# Autodesk Inventor assembly: アームアセンブリ
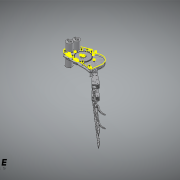
[picture p0: Inventor's stored thumbnail of the model, 180x180]
Saved by Autodesk Inventor 2020 (Build 240168000, 168)
## iProperties
Created: 2019-12-03
Part Number: アームアセンブリ
Material: 一般
Document SubType Name: Assembly
Designer: tanjihayato
Mass: 763.38 g
Surface Area: 1766.69 cm^2
Volume: 307.552 cm^3
Density: 2.48212 g/cm^3
Author: tanjihayato
## Documents named in this file (28)
- \\Mac\Home\Documents\Inventor\2019お遊び機体\アームアセンブリ.iam
- \\Mac\Home\Documents\Inventor\2019お遊び機体\アーム右フレーム.ipt
- \\Mac\Home\Documents\Inventor\2019お遊び機体\アーム真ん中フレーム.ipt
- \\Mac\Home\Documents\Inventor\2019お遊び機体\スペーサ　m3-l12.ipt
- \\Mac\Home\Documents\Inventor\2019お遊び機体\モーター(形だけ).ipt
- \\Mac\Home\Documents\Inventor\2019お遊び機体\キャップボルトM3×8.ipt
- \\Mac\Home\Documents\Inventor\2019お遊び機体\m1 64.ipt
- \\Mac\Home\Documents\Inventor\2019お遊び機体\m2z10はめあい.ipt
- \\Mac\Home\Documents\Inventor\2019お遊び機体\アーム左フレーム.ipt
- \\Mac\Home\Documents\Inventor\2019お遊び機体\スペーサ　m4-l35.ipt
- \\Mac\Home\Documents\Inventor\2019お遊び機体\スペーサ　m4-l18.ipt
- \\Mac\Home\Documents\Inventor\2019お遊び機体\アーム駆動抑え.ipt
- \\Mac\Home\Documents\Inventor\2019お遊び機体\フランジブッシュ　d6-D8-l5-h12.ipt
- \\Mac\Home\Documents\Inventor\2019お遊び機体\スペーサ　m3-l6.ipt
- \\Mac\Home\Documents\Inventor\2019お遊び機体\アーム最終段円盤.ipt
- \\Mac\Home\Documents\Inventor\2019お遊び機体\アーム中間節.ipt
- \\Mac\Home\Documents\Inventor\2019お遊び機体\アーム揺動節.ipt
- \\Mac\Home\Documents\Inventor\2019お遊び機体\アーム中間節_MIR.ipt
- \\Mac\Home\Documents\Inventor\2019お遊び機体\シールド殺し.ipt
- \\Mac\Home\Documents\Inventor\2019お遊び機体\ロッド.ipt
- \\Mac\Home\Documents\Inventor\2019お遊び機体\シールド殺し_MIR.ipt
- \\Mac\Home\Documents\Inventor\2019お遊び機体\ロッド根本.ipt
- \\Mac\Home\Documents\Inventor\2019お遊び機体\ロッド根本２.ipt
- \\Mac\Home\Documents\Inventor\2019お遊び機体\ロッド根本２_MIR.ipt
- \\Mac\Home\Documents\Inventor\2019お遊び機体\ロッド根本_MIR.ipt
- \\Mac\Home\Documents\Inventor\2019お遊び機体\スペーサ　m3-l14.ipt
- \\Mac\Home\Documents\Inventor\2019お遊び機体\アダプター.ipt
- \\Mac\Home\Documents\Inventor\2019お遊び機体\アダプター_MIR.ipt
## Components (74 placed, 27 different names)
1. アーム右フレーム:1 — 挿入:10, メイト:1, 挿入:12, 挿入:14, 挿入:15, 挿入:16, 挿入:17, 挿入:18, 挿入:19, 挿入:20, 挿入:21, 挿入:22, 挿入:23, 挿入:33, 挿入:34, 挿入:35
2. アーム真ん中フレーム:1 — 挿入:1, 挿入:2, 挿入:3, 挿入:4, 挿入:5, 挿入:6, 挿入:7, 挿入:8, 挿入:9, 挿入:11, 挿入:13, 挿入:24, 挿入:25, 挿入:26, 挿入:27, 挿入:28, 挿入:29, 挿入:30, 挿入:31, 挿入:32, 挿入:37, 挿入:41
3. スペーサ　m3-l12:1 — 挿入:6
4. スペーサ　m3-l12:2 — 挿入:9
5. スペーサ　m3-l12:3 — 挿入:4, 挿入:10
6. スペーサ　m3-l12:4 — 挿入:8
7. スペーサ　m3-l12:5 — 挿入:5, メイト:1
8. スペーサ　m3-l12:6 — 挿入:7
9. スペーサ　m3-l12:7 — 挿入:1
10. スペーサ　m3-l12:8 — 挿入:3
11. スペーサ　m3-l12:9 — 挿入:2
12. モーター(形だけ):1 — 挿入:11
13. モーター(形だけ):2 — 挿入:14
14. モーター(形だけ):3 — 挿入:12
15. モーター(形だけ):4 — 挿入:13
16. キャップボルトM3×8:1 — 挿入:17
17. キャップボルトM3×8:2 — 挿入:15
18. キャップボルトM3×8:3 — 挿入:20
19. キャップボルトM3×8:4 — 挿入:18
20. キャップボルトM3×8:5 — 挿入:22
21. キャップボルトM3×8:6 — 挿入:19
22. キャップボルトM3×8:7 — 挿入:28
23. キャップボルトM3×8:8 — 挿入:27
24. キャップボルトM3×8:9 — 挿入:24
25. キャップボルトM3×8:10 — 挿入:25
26. キャップボルトM3×8:11 — 挿入:29
27. キャップボルトM3×8:12 — 挿入:26
28. キャップボルトM3×8:13 — 挿入:30
29. キャップボルトM3×8:14 — 挿入:23
30. キャップボルトM3×8:15 — 挿入:31
31. キャップボルトM3×8:16 — 挿入:21
32. キャップボルトM3×8:17 — 挿入:32
33. キャップボルトM3×8:18 — 挿入:16
34. m1 64:1 — フラッシュ:1, メイト:2, メイト:3
35. m2z10はめあい:1 — フラッシュ:1, メイト:2, メイト:3, 挿入:33
36. アーム左フレーム:1 — 挿入:36, メイト:4, 挿入:38
37. スペーサ　m4-l35:1 — 挿入:34, 挿入:36
38. スペーサ　m4-l35:2 — 挿入:35, メイト:4
39. スペーサ　m4-l18:1 — 挿入:37, メイト:7
40. アーム駆動抑え:1 — 挿入:39, メイト:5
41. フランジブッシュ　d6-D8-l5-h12:1 — 挿入:38, 挿入:40
42. スペーサ　m3-l6:1 — 挿入:39, 挿入:40
43. アーム最終段円盤:1 — 挿入:41, メイト:5, 挿入:44
44. アーム中間節:1 — 挿入:42, 挿入:43, メイト:6, 挿入:44, 挿入:73, メイト:20
45. アーム揺動節:1 — 挿入:42, メイト:7
46. アーム中間節_MIR:1 — 挿入:43, メイト:6, 挿入:74, メイト:21
47. シールド殺し:2 — 挿入:45, メイト:8
48. ロッド:1 — 挿入:46, メイト:9, 挿入:77, メイト:24, 挿入:79
49. ロッド:2 — 挿入:45, メイト:8, 挿入:76, メイト:23, 挿入:78
50. シールド殺し_MIR:1 — 挿入:46, メイト:9
51. ロッド根本:1 — 挿入:55, 挿入:56, 挿入:57, 挿入:72, メイト:19
52. ロッド根本２:1 — 挿入:54, 挿入:77, メイト:24
53. ロッド根本２:4 — 挿入:53, 挿入:76, メイト:23
54. ロッド根本:4 — 挿入:62, メイト:15
55. ロッド根本２_MIR:1 — 挿入:51, 挿入:67, 挿入:68, 挿入:78
56. ロッド根本２_MIR:2 — 挿入:52, 挿入:65, 挿入:66, 挿入:79
57. フランジブッシュ　d6-D8-l5-h12:2 — 挿入:51, 挿入:64
58. フランジブッシュ　d6-D8-l5-h12:3 — 挿入:53
59. フランジブッシュ　d6-D8-l5-h12:4 — 挿入:52, 挿入:63
60. フランジブッシュ　d6-D8-l5-h12:5 — 挿入:54
61. ロッド根本_MIR:1 — 挿入:58, メイト:14, 挿入:63
62. ロッド根本_MIR:2 — 挿入:59, 挿入:60, 挿入:61, 挿入:64, 挿入:75, メイト:22
63. スペーサ　m3-l14:1 — 挿入:55, 挿入:58
64. スペーサ　m3-l14:2 — 挿入:56
65. スペーサ　m3-l14:3 — 挿入:57, メイト:14
66. スペーサ　m3-l14:4 — 挿入:59
67. スペーサ　m3-l14:5 — 挿入:60, 挿入:62
68. スペーサ　m3-l14:6 — 挿入:61, メイト:15
69. スペーサ　m3-l6:2 — 挿入:66
70. スペーサ　m3-l6:3 — 挿入:67
71. スペーサ　m3-l6:4 — 挿入:65
72. スペーサ　m3-l6:5 — 挿入:68
73. アダプター:1 — 挿入:72, メイト:19, 挿入:73, メイト:20
74. アダプター_MIR:1 — 挿入:74, メイト:21, 挿入:75, メイト:22
## Relationships (90: Insert 72, Mate 17, Flush 1)
- 挿入:1 [Insert]: アーム真ん中フレーム:1 ↔ スペーサ　m3-l12:7
- 挿入:2 [Insert]: アーム真ん中フレーム:1 ↔ スペーサ　m3-l12:9
- 挿入:3 [Insert]: アーム真ん中フレーム:1 ↔ スペーサ　m3-l12:8
- 挿入:4 [Insert]: アーム真ん中フレーム:1 ↔ スペーサ　m3-l12:3
- 挿入:5 [Insert]: アーム真ん中フレーム:1 ↔ スペーサ　m3-l12:5
- 挿入:6 [Insert]: アーム真ん中フレーム:1 ↔ スペーサ　m3-l12:1
- 挿入:7 [Insert]: アーム真ん中フレーム:1 ↔ スペーサ　m3-l12:6
- 挿入:8 [Insert]: アーム真ん中フレーム:1 ↔ スペーサ　m3-l12:4
- 挿入:9 [Insert]: アーム真ん中フレーム:1 ↔ スペーサ　m3-l12:2
- 挿入:10 [Insert]: アーム右フレーム:1 ↔ スペーサ　m3-l12:3
- メイト:1 [Mate]: アーム右フレーム:1 ↔ スペーサ　m3-l12:5
- 挿入:11 [Insert]: アーム真ん中フレーム:1 ↔ モーター(形だけ):1
- 挿入:12 [Insert]: アーム右フレーム:1 ↔ モーター(形だけ):3
- 挿入:13 [Insert]: アーム真ん中フレーム:1 ↔ モーター(形だけ):4
- 挿入:14 [Insert]: アーム右フレーム:1 ↔ モーター(形だけ):2
- 挿入:15 [Insert]: アーム右フレーム:1 ↔ キャップボルトM3×8:2
- 挿入:16 [Insert]: アーム右フレーム:1 ↔ キャップボルトM3×8:18
- 挿入:17 [Insert]: アーム右フレーム:1 ↔ キャップボルトM3×8:1
- 挿入:18 [Insert]: アーム右フレーム:1 ↔ キャップボルトM3×8:4
- 挿入:19 [Insert]: アーム右フレーム:1 ↔ キャップボルトM3×8:6
- 挿入:20 [Insert]: アーム右フレーム:1 ↔ キャップボルトM3×8:3
- 挿入:21 [Insert]: アーム右フレーム:1 ↔ キャップボルトM3×8:16
- 挿入:22 [Insert]: アーム右フレーム:1 ↔ キャップボルトM3×8:5
- 挿入:23 [Insert]: アーム右フレーム:1 ↔ キャップボルトM3×8:14
- 挿入:24 [Insert]: アーム真ん中フレーム:1 ↔ キャップボルトM3×8:9
- 挿入:25 [Insert]: アーム真ん中フレーム:1 ↔ キャップボルトM3×8:10
- 挿入:26 [Insert]: アーム真ん中フレーム:1 ↔ キャップボルトM3×8:12
- 挿入:27 [Insert]: アーム真ん中フレーム:1 ↔ キャップボルトM3×8:8
- 挿入:28 [Insert]: アーム真ん中フレーム:1 ↔ キャップボルトM3×8:7
- 挿入:29 [Insert]: アーム真ん中フレーム:1 ↔ キャップボルトM3×8:11
- 挿入:30 [Insert]: アーム真ん中フレーム:1 ↔ キャップボルトM3×8:13
- 挿入:31 [Insert]: アーム真ん中フレーム:1 ↔ キャップボルトM3×8:15
- 挿入:32 [Insert]: アーム真ん中フレーム:1 ↔ キャップボルトM3×8:17
- フラッシュ:1 [Flush]: m1 64:1 ↔ m2z10はめあい:1
- メイト:2 [Mate]: m1 64:1 ↔ m2z10はめあい:1
- メイト:3 [Mate]: m1 64:1 ↔ m2z10はめあい:1
- 挿入:33 [Insert] (1 mm): アーム右フレーム:1 ↔ m2z10はめあい:1
- 挿入:34 [Insert]: アーム右フレーム:1 ↔ スペーサ　m4-l35:1
- 挿入:35 [Insert]: アーム右フレーム:1 ↔ スペーサ　m4-l35:2
- 挿入:36 [Insert]: アーム左フレーム:1 ↔ スペーサ　m4-l35:1
- メイト:4 [Mate]: アーム左フレーム:1 ↔ スペーサ　m4-l35:2
- 挿入:37 [Insert]: アーム真ん中フレーム:1 ↔ スペーサ　m4-l18:1
- 挿入:38 [Insert]: アーム左フレーム:1 ↔ フランジブッシュ　d6-D8-l5-h12:1
- 挿入:39 [Insert]: アーム駆動抑え:1 ↔ スペーサ　m3-l6:1
- 挿入:40 [Insert]: フランジブッシュ　d6-D8-l5-h12:1 ↔ スペーサ　m3-l6:1
- 挿入:41 [Insert] (0.5 mm): アーム真ん中フレーム:1 ↔ アーム最終段円盤:1
- メイト:5 [Mate]: アーム駆動抑え:1 ↔ アーム最終段円盤:1
- 挿入:42 [Insert] (0.5 mm): アーム中間節:1 ↔ アーム揺動節:1
- 挿入:43 [Insert]: アーム中間節:1 ↔ アーム中間節_MIR:1
- メイト:6 [Mate]: アーム中間節:1 ↔ アーム中間節_MIR:1
- メイト:7 [Mate]: スペーサ　m4-l18:1 ↔ アーム揺動節:1
- 挿入:44 [Insert] (8 mm): アーム最終段円盤:1 ↔ アーム中間節:1
- 挿入:45 [Insert]: シールド殺し:2 ↔ ロッド:2
- メイト:8 [Mate]: シールド殺し:2 ↔ ロッド:2
- 挿入:46 [Insert]: ロッド:1 ↔ シールド殺し_MIR:1
- メイト:9 [Mate]: ロッド:1 ↔ シールド殺し_MIR:1
- 挿入:51 [Insert]: ロッド根本２_MIR:1 ↔ フランジブッシュ　d6-D8-l5-h12:2
- 挿入:52 [Insert]: ロッド根本２_MIR:2 ↔ フランジブッシュ　d6-D8-l5-h12:4
- 挿入:53 [Insert]: ロッド根本２:4 ↔ フランジブッシュ　d6-D8-l5-h12:3
- 挿入:54 [Insert]: ロッド根本２:1 ↔ フランジブッシュ　d6-D8-l5-h12:5
- 挿入:55 [Insert]: ロッド根本:1 ↔ スペーサ　m3-l14:1
- 挿入:56 [Insert]: ロッド根本:1 ↔ スペーサ　m3-l14:2
- 挿入:57 [Insert]: ロッド根本:1 ↔ スペーサ　m3-l14:3
- 挿入:58 [Insert]: ロッド根本_MIR:1 ↔ スペーサ　m3-l14:1
- メイト:14 [Mate]: ロッド根本_MIR:1 ↔ スペーサ　m3-l14:3
- 挿入:59 [Insert]: ロッド根本_MIR:2 ↔ スペーサ　m3-l14:4
- 挿入:60 [Insert]: ロッド根本_MIR:2 ↔ スペーサ　m3-l14:5
- 挿入:61 [Insert]: ロッド根本_MIR:2 ↔ スペーサ　m3-l14:6
- 挿入:62 [Insert]: ロッド根本:4 ↔ スペーサ　m3-l14:5
- メイト:15 [Mate]: ロッド根本:4 ↔ スペーサ　m3-l14:6
- 挿入:63 [Insert]: フランジブッシュ　d6-D8-l5-h12:4 ↔ ロッド根本_MIR:1
- 挿入:64 [Insert]: フランジブッシュ　d6-D8-l5-h12:2 ↔ ロッド根本_MIR:2
- 挿入:65 [Insert]: ロッド根本２_MIR:2 ↔ スペーサ　m3-l6:4
- 挿入:66 [Insert]: ロッド根本２_MIR:2 ↔ スペーサ　m3-l6:2
- 挿入:67 [Insert]: ロッド根本２_MIR:1 ↔ スペーサ　m3-l6:3
- 挿入:68 [Insert]: ロッド根本２_MIR:1 ↔ スペーサ　m3-l6:5
- 挿入:72 [Insert]: ロッド根本:1 ↔ アダプター:1
- メイト:19 [Mate]: ロッド根本:1 ↔ アダプター:1
- 挿入:73 [Insert]: アーム中間節:1 ↔ アダプター:1
- メイト:20 [Mate]: アーム中間節:1 ↔ アダプター:1
- 挿入:74 [Insert]: アーム中間節_MIR:1 ↔ アダプター_MIR:1
- メイト:21 [Mate]: アーム中間節_MIR:1 ↔ アダプター_MIR:1
- 挿入:75 [Insert]: ロッド根本_MIR:2 ↔ アダプター_MIR:1
- メイト:22 [Mate]: ロッド根本_MIR:2 ↔ アダプター_MIR:1
- 挿入:76 [Insert]: ロッド:2 ↔ ロッド根本２:4
- メイト:23 [Mate]: ロッド:2 ↔ ロッド根本２:4
- 挿入:77 [Insert]: ロッド:1 ↔ ロッド根本２:1
- メイト:24 [Mate]: ロッド:1 ↔ ロッド根本２:1
- 挿入:78 [Insert]: ロッド:2 ↔ ロッド根本２_MIR:1
- 挿入:79 [Insert]: ロッド:1 ↔ ロッド根本２_MIR:2
